# Autodesk Inventor assembly: Tensionador-4-Cabos
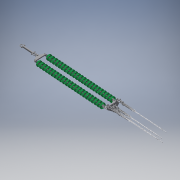
[picture p0: Inventor's stored thumbnail of the model, 180x180]
Saved by Autodesk Inventor 2018 (Build 220112000, 112)
## iProperties
Created: 2021-04-28
Part Number: Tensionador-4-Cabos
Document SubType Name: Assembly
Designer: l01767
Author: l01767
## Documents named in this file (10)
- F:\Projetos\TAESA\Modelo 3D - Tensionadores e Suspensão\Tensionador\Tensionador-4-Cabos.iam
- F:\Projetos\TAESA\Modelo 3D - Tensionadores e Suspensão\Tensionador\gpghmb32.iam
- F:\Projetos\TAESA\Modelo 3D - Tensionadores e Suspensão\Tensionador\Link_Principal.ipt
- F:\Projetos\TAESA\Modelo 3D - Tensionadores e Suspensão\Tensionador\Espacador_Delta.ipt
- F:\Projetos\TAESA\Modelo 3D - Tensionadores e Suspensão\Tensionador\Clevis-Bola_Curto.ipt
- F:\Projetos\TAESA\Modelo 3D - Tensionadores e Suspensão\Tensionador\Bolted Connection1.iam
- F:\Projetos\TAESA\Modelo 3D - Tensionadores e Suspensão\Tensionador\U300B.iam
- F:\Projetos\TAESA\Modelo 3D - Tensionadores e Suspensão\Tensionador\Clevis-Socket.iam
- F:\Projetos\TAESA\Modelo 3D - Tensionadores e Suspensão\Tensionador\Balancim_4-Cabos_Modelo2.ipt
- F:\Projetos\TAESA\Modelo 3D - Tensionadores e Suspensão\Tensionador\OPGW Tension set.iam
## Components (70 placed, 9 different names)
1. gpghmb32:1 [sub-assembly] — Mate:1, Mate:2, Flush:1, Mate:3, Mate:4, Mate:6
2. gpghmb32:2 [sub-assembly] — Mate:5, Mate:7, Flush:2, Flush:11, Flush:10, Tangent:1
3. Link_Principal:1 — Mate:1, Mate:4, Mate:5, Mate:6, Mate:7, Flush:2
4. gpghmb32:3 [sub-assembly] — Flush:11, Flush:10, Tangent:1, Mate:8, Mate:9, Mate:10
5. Espacador_Delta:1 — Mate:8, Mate:9, Mate:10, Mate:11, Angle:1, Mate:12
6. Clevis-Socket:1 [sub-assembly] — Mate:23, Mate:24, Flush:30, Mate:30
7. Clevis-Socket:3 [sub-assembly] — Mate:27, Mate:28, Mate:29
8. Balancim_4-Cabos_Modelo2:1 — Flush:30, Mate:29, Mate:30, Mate:31, Mate:32, Mate:33, Mate:34, Mate:35, Mate:36, Mate:37, Angle:3, Angle:4, Angle:5, Angle:6, Mate:46
9. gpghmb32:4 [sub-assembly] — Mate:31, Mate:35, Angle:3, Mate:40, Mate:41, Tangent:2
10. gpghmb32:5 [sub-assembly] — Mate:32, Mate:36, Angle:4, Mate:42, Mate:43, Tangent:4
11. gpghmb32:6 [sub-assembly] — Mate:33, Angle:5, Mate:38, Mate:39, Mate:46, Tangent:5
12. gpghmb32:7 [sub-assembly] — Mate:34, Mate:37, Angle:6, Mate:44, Mate:45, Tangent:3
13. gpghmb32:8 [sub-assembly] — Mate:38, Mate:39, Tangent:5, Mate:47, Flush:31
14. gpghmb32:9 [sub-assembly] — Mate:44, Mate:45, Tangent:3, Mate:50
15. gpghmb32:10 [sub-assembly] — Mate:40, Mate:41, Tangent:2, Mate:49, Flush:32
16. gpghmb32:11 [sub-assembly] — Mate:42, Mate:43, Tangent:4, Mate:48
17. OPGW Tension set:1 [sub-assembly] — Mate:47, Flush:31
18. OPGW Tension set:2 [sub-assembly] — Mate:48
19. OPGW Tension set:3 [sub-assembly] — Mate:49, Flush:32
20. OPGW Tension set:4 [sub-assembly] — Mate:50
21. Clevis-Bola_Curto:1 — Mate:11, Angle:1, Mate:12, Mate:13, Mate:14, Mate:15, Mate:16, Angle:2
22. Bolted Connection:1 [sub-assembly] — Mate:13, Mate:14
23. Clevis-Bola_Curto:2
24. Bolted Connection:2 [sub-assembly]
25. U300B:1 [sub-assembly] — Mate:15, Mate:16, Angle:2
26. U300B:2 [sub-assembly]
27. U300B:3 [sub-assembly]
28. U300B:4 [sub-assembly]
29. U300B:5 [sub-assembly]
30. U300B:6 [sub-assembly]
31. U300B:7 [sub-assembly]
32. U300B:8 [sub-assembly]
33. U300B:9 [sub-assembly]
34. U300B:10 [sub-assembly]
35. U300B:11 [sub-assembly]
36. U300B:12 [sub-assembly]
37. U300B:13 [sub-assembly]
38. U300B:14 [sub-assembly]
39. U300B:15 [sub-assembly]
40. U300B:16 [sub-assembly]
41. U300B:17 [sub-assembly]
42. U300B:18 [sub-assembly]
43. U300B:19 [sub-assembly]
44. U300B:20 [sub-assembly]
45. U300B:21 [sub-assembly]
46. U300B:22 [sub-assembly]
47. U300B:23 [sub-assembly] — Mate:23, Mate:24
48. U300B:24 [sub-assembly]
49. U300B:25 [sub-assembly]
50. U300B:26 [sub-assembly]
51. U300B:27 [sub-assembly]
52. U300B:28 [sub-assembly]
53. U300B:29 [sub-assembly]
54. U300B:30 [sub-assembly]
55. U300B:31 [sub-assembly]
56. U300B:32 [sub-assembly]
57. U300B:33 [sub-assembly]
58. U300B:34 [sub-assembly]
59. U300B:35 [sub-assembly]
60. U300B:36 [sub-assembly]
61. U300B:37 [sub-assembly]
62. U300B:38 [sub-assembly]
63. U300B:39 [sub-assembly]
64. U300B:40 [sub-assembly]
65. U300B:41 [sub-assembly]
66. U300B:42 [sub-assembly]
67. U300B:43 [sub-assembly]
68. U300B:44 [sub-assembly]
69. U300B:45 [sub-assembly]
70. U300B:46 [sub-assembly] — Mate:27, Mate:28
## Component patterns: (2 elements, first: Clevis-Bola_Curto:1 + Bolted Connection:1), (23 elements, first: U300B:1), Component Pattern 1:2 (23 elements)
## Relationships (60: Mate 42, Flush 7, Angle 6, Tangent 5)
- Mate:1: gpghmb32:1 ↔ Link_Principal:1
- Mate:2: gpghmb32:1
- Flush:1: gpghmb32:1
- Mate:3: gpghmb32:1
- Mate:4: gpghmb32:1 ↔ Link_Principal:1
- Mate:5: gpghmb32:2 ↔ Link_Principal:1
- Mate:6: gpghmb32:1 ↔ Link_Principal:1
- Mate:7: gpghmb32:2 ↔ Link_Principal:1
- Flush:2: gpghmb32:2 ↔ Link_Principal:1
- Flush:11: gpghmb32:2 ↔ gpghmb32:3
- Flush:10: gpghmb32:2 ↔ gpghmb32:3
- Tangent:1: gpghmb32:2 ↔ gpghmb32:3
- Mate:8: gpghmb32:3 ↔ Espacador_Delta:1
- Mate:9: gpghmb32:3 ↔ Espacador_Delta:1
- Mate:10: gpghmb32:3 ↔ Espacador_Delta:1
- Mate:11: Espacador_Delta:1 ↔ Clevis-Bola_Curto:1
- Angle:1 (180 deg): Espacador_Delta:1 ↔ Clevis-Bola_Curto:1
- Mate:12: Espacador_Delta:1 ↔ Clevis-Bola_Curto:1
- Mate:13: Clevis-Bola_Curto:1 ↔ Bolted Connection:1
- Mate:14: Clevis-Bola_Curto:1 ↔ Bolted Connection:1
- Mate:15: Clevis-Bola_Curto:1 ↔ U300B:1
- Mate:16 (5 mm): Clevis-Bola_Curto:1 ↔ U300B:1
- Angle:2 (0 deg): Clevis-Bola_Curto:1 ↔ U300B:1
- Mate:23: Clevis-Socket:1 ↔ U300B:23
- Mate:24 (15 mm): Clevis-Socket:1 ↔ U300B:23
- Mate:27: Clevis-Socket:3 ↔ U300B:46
- Mate:28 (15 mm): Clevis-Socket:3 ↔ U300B:46
- Flush:30: Clevis-Socket:1 ↔ Balancim_4-Cabos_Modelo2:1
- Mate:29: Clevis-Socket:3 ↔ Balancim_4-Cabos_Modelo2:1
- Mate:30: Clevis-Socket:1 ↔ Balancim_4-Cabos_Modelo2:1
- Mate:31: Balancim_4-Cabos_Modelo2:1 ↔ gpghmb32:4
- Mate:32: Balancim_4-Cabos_Modelo2:1 ↔ gpghmb32:5
- Mate:33: Balancim_4-Cabos_Modelo2:1 ↔ gpghmb32:6
- Mate:34: Balancim_4-Cabos_Modelo2:1 ↔ gpghmb32:7
- Mate:35: Balancim_4-Cabos_Modelo2:1 ↔ gpghmb32:4
- Mate:36: Balancim_4-Cabos_Modelo2:1 ↔ gpghmb32:5
- Mate:37: Balancim_4-Cabos_Modelo2:1 ↔ gpghmb32:7
- Angle:3 (0 deg): Balancim_4-Cabos_Modelo2:1 ↔ gpghmb32:4
- Angle:4 (0 deg): Balancim_4-Cabos_Modelo2:1 ↔ gpghmb32:5
- Angle:5 (0 deg): Balancim_4-Cabos_Modelo2:1 ↔ gpghmb32:6
- Angle:6 (0 deg): Balancim_4-Cabos_Modelo2:1 ↔ gpghmb32:7
- Mate:38: gpghmb32:6 ↔ gpghmb32:8
- Mate:39: gpghmb32:6 ↔ gpghmb32:8
- Mate:40: gpghmb32:4 ↔ gpghmb32:10
- Mate:41: gpghmb32:4 ↔ gpghmb32:10
- Mate:42: gpghmb32:5 ↔ gpghmb32:11
- Mate:43: gpghmb32:5 ↔ gpghmb32:11
- Mate:44: gpghmb32:7 ↔ gpghmb32:9
- Mate:45: gpghmb32:7 ↔ gpghmb32:9
- Mate:46: Balancim_4-Cabos_Modelo2:1 ↔ gpghmb32:6
- Tangent:2: gpghmb32:4 ↔ gpghmb32:10
- Tangent:3: gpghmb32:7 ↔ gpghmb32:9
- Tangent:4: gpghmb32:5 ↔ gpghmb32:11
- Tangent:5: gpghmb32:6 ↔ gpghmb32:8
- Mate:47: gpghmb32:8 ↔ OPGW Tension set:1
- Mate:48: gpghmb32:11 ↔ OPGW Tension set:2
- Mate:49: gpghmb32:10 ↔ OPGW Tension set:3
- Mate:50: gpghmb32:9 ↔ OPGW Tension set:4
- Flush:31: gpghmb32:8 ↔ OPGW Tension set:1
- Flush:32: gpghmb32:10 ↔ OPGW Tension set:3
